# Autodesk Inventor assembly: Assembly2
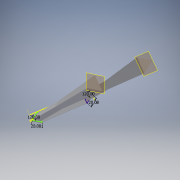
[picture p0: Inventor's stored thumbnail of the model, 180x180]
Saved by Autodesk Inventor 2016 (Build 200138000, 138)
## iProperties
Created: 2015-12-05
Part Number: Assembly2
Document SubType Name: Assembly
Designer: acd
Author: acd
## Documents named in this file (5)
- C:\Users\acd\Google Drive\OTHER\MY GRE!\PORTFOLIO\Harp#\Assembly2.iam
- C:\Users\acd\Google Drive\OTHER\MY GRE!\PORTFOLIO\Harp#\pillar.ipt
- C:\Users\acd\Google Drive\OTHER\MY GRE!\PORTFOLIO\Harp#\top.ipt
- C:\Users\acd\Google Drive\OTHER\MY GRE!\PORTFOLIO\Harp#\connector.ipt
- C:\Users\acd\Google Drive\OTHER\MY GRE!\PORTFOLIO\Harp#\mirror.ipt
## Components (6 placed, 4 different names)
1. pillar:1 — Mate:1, Mate:3, Mate:15
2. pillar:2 — Mate:2, Mate:4, Mate:14
3. top:1 — Mate:1, Mate:2, Mate:3, Mate:4, Mate:5, Mate:6, Mate:7, Mate:8, Mate:9, Mate:10, Mate:14, Mate:15
4. connector:1 — Mate:5, Mate:6, Mate:7, Mate:12
5. connector:2 — Mate:8, Mate:9, Mate:10, Mate:11, Mate:16
6. mirror:1 — Mate:11, Mate:12, Mate:16
## Relationships (15: Mate 15)
- Mate:1: pillar:1 ↔ top:1
- Mate:2: pillar:2 ↔ top:1
- Mate:3: pillar:1 ↔ top:1
- Mate:4: pillar:2 ↔ top:1
- Mate:5: top:1 ↔ connector:1
- Mate:6: top:1 ↔ connector:1
- Mate:7: top:1 ↔ connector:1
- Mate:8: top:1 ↔ connector:2
- Mate:9: top:1 ↔ connector:2
- Mate:10: top:1 ↔ connector:2
- Mate:11: connector:2 ↔ mirror:1
- Mate:12: connector:1 ↔ mirror:1
- Mate:14: pillar:2 ↔ top:1
- Mate:15: pillar:1 ↔ top:1
- Mate:16: connector:2 ↔ mirror:1
